# Autodesk Inventor assembly: Microbot
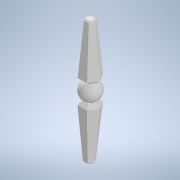
[picture p0: Inventor's stored thumbnail of the model, 180x180]
Saved by Autodesk Inventor 2022 (Build 260153000, 153)
## iProperties
Created: 2022-02-07
Part Number: Microbot
Document SubType Name: Assembly
Designer: mogje
Author: mogje
## Documents named in this file (3)
- D:\Program Files (x86)\Autodesk Inventor\Projects\Microbots\Microbot.iam
- D:\Program Files (x86)\Autodesk Inventor\Projects\Microbots\Connector.ipt
- D:\Program Files (x86)\Autodesk Inventor\Projects\Microbots\Microbot Half.ipt
## Components (3 placed, 2 different names)
1. Connector:1 — Mate:1, Mate:2, Mate:3, Mate:4
2. Microbot Half:1 — Mate:1, Mate:2
3. Microbot Half:2 — Mate:3, Mate:4
## Relationships (4: Mate 4)
- Mate:1: Connector:1 ↔ Microbot Half:1
- Mate:2: Connector:1 ↔ Microbot Half:1
- Mate:3: Connector:1 ↔ Microbot Half:2
- Mate:4: Connector:1 ↔ Microbot Half:2
